# Autodesk Inventor assembly: Mind
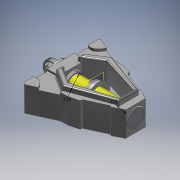
[picture p0: Inventor's stored thumbnail of the model, 180x180]
Saved by Autodesk Inventor 2019 (Build 230136000, 136)
## iProperties
Created: 2019-05-15
Part Number: Mind
Document SubType Name: Assembly
Designer: Jorian Brusind
Author: Jorian Brusind
## Documents named in this file (4)
- C:\Users\Jorian Brusind\Documents\GitHub\PersonalProjects\Inventor Projects\Infinity\Mind.iam
- C:\Users\Jorian Brusind\Documents\GitHub\PersonalProjects\Inventor Projects\Infinity\Yellow.ipt
- C:\Users\Jorian Brusind\Documents\GitHub\PersonalProjects\Inventor Projects\Infinity\Holder.ipt
- C:\Users\Jorian Brusind\Documents\GitHub\PersonalProjects\Inventor Projects\Infinity\EndCap.ipt
## Components (4 placed, 3 different names)
1. Yellow:1 — Mate:1, Mate:5
2. Holder:1 — Mate:1, Mate:2, Mate:3, Mate:4, Flush:1
3. EndCap:1 — Mate:4, Flush:1, Mate:5
4. EndCap:2 — Mate:2, Mate:3
## Relationships (6: Mate 5, Flush 1)
- Mate:1: Yellow:1 ↔ Holder:1
- Mate:2: Holder:1 ↔ EndCap:2
- Mate:3: Holder:1 ↔ EndCap:2
- Mate:4: Holder:1 ↔ EndCap:1
- Flush:1: Holder:1 ↔ EndCap:1
- Mate:5: Yellow:1 ↔ EndCap:1
